# Autodesk Inventor assembly: PegAssembly
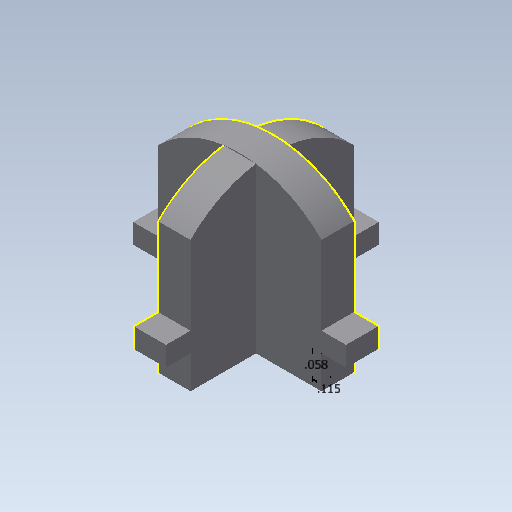
[picture p0: Inventor's stored thumbnail of the model, 512x512]
Saved by Autodesk Inventor 2020.1 (Build 241239000, 239)
## iProperties
Created: 2019-10-29
Part Number: PegAssembly
Document SubType Name: Assembly
Designer: ls
Author: ls
## Documents named in this file (3)
- C:\Users\amirs\OneDrive - UC San Diego\college\freshman year\MAE 3\robot\drive train\PegAssembly (1).iam
- C:\Users\amirs\OneDrive - UC San Diego\college\freshman year\MAE 3\robot\drive train\TopPegCor.ipt
- C:\Users\amirs\OneDrive - UC San Diego\college\freshman year\MAE 3\robot\drive train\BottomPegCor.ipt
## Components (2 placed, 2 different names)
1. TopPegCor:1 — Mate:1, Mate:2, Mate:3
2. BottomPegCor:1 — Mate:1, Mate:2, Mate:3
## Relationships (3: Mate 3)
- Mate:1: TopPegCor:1 ↔ BottomPegCor:1
- Mate:2: TopPegCor:1 ↔ BottomPegCor:1
- Mate:3: TopPegCor:1 ↔ BottomPegCor:1
